# Autodesk Inventor assembly: gyro asmb
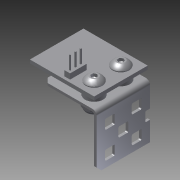
[picture p0: Inventor's stored thumbnail of the model, 180x180]
Saved by Autodesk Inventor 2014 SP1 (Build 180222100, 222)
## iProperties
Created: 2014-03-19
Part Number: gyro asmb
Document SubType Name: Assembly
Designer: Ryan
Author: Ryan
## Documents named in this file (5)
- C:\Users\Ryan\Desktop\sw\toss up 4th robot\tower\gyro asmb.iam
- C:\Users\Ryan\Desktop\sw\lib\Aperture VEX CAD Library\Electronics\gyro\gyro.ipt
- C:\Users\Ryan\Desktop\sw\lib\Aperture VEX CAD Library\Metal\L Bar\2 x 2.ipt
- C:\Users\Ryan\Desktop\sw\lib\Aperture VEX CAD Library\Hardware\8-32\8-32_.375.ipt
- C:\Users\Ryan\Desktop\sw\lib\Aperture VEX CAD Library\Hardware\8-32\8-32 nylock.ipt
## Components (6 placed, 4 different names)
1. gyro:1 — Mate:1, Mate:2, Mate:3, Mate:4, Mate:5, Mate:6, Mate:7, Mate:8
2. 2 x 2:1 — Mate:1, Mate:2, Mate:3, Mate:4, Mate:9, Mate:12
3. 8-32_.375:1 — Mate:5, Mate:6, Mate:10
4. 8-32_.375:2 — Mate:7, Mate:8, Mate:11
5. 8-32 nylock:1 — Mate:9, Mate:10
6. 8-32 nylock:2 — Mate:11, Mate:12
## Relationships (12: Mate 12)
- Mate:1: gyro:1 ↔ 2 x 2:1
- Mate:2 (2.3114 mm): gyro:1 ↔ 2 x 2:1
- Mate:3 (2.3114 mm): gyro:1 ↔ 2 x 2:1
- Mate:4 (2.3114 mm): gyro:1 ↔ 2 x 2:1
- Mate:5: gyro:1 ↔ 8-32_.375:1
- Mate:6: gyro:1 ↔ 8-32_.375:1
- Mate:7: gyro:1 ↔ 8-32_.375:2
- Mate:8: gyro:1 ↔ 8-32_.375:2
- Mate:9: 2 x 2:1 ↔ 8-32 nylock:1
- Mate:10: 8-32_.375:1 ↔ 8-32 nylock:1
- Mate:11: 8-32_.375:2 ↔ 8-32 nylock:2
- Mate:12: 2 x 2:1 ↔ 8-32 nylock:2
## Named parameters: q = 2.3114 mm
